# Autodesk Inventor assembly: Glue Stamp Staging Plate Assembly
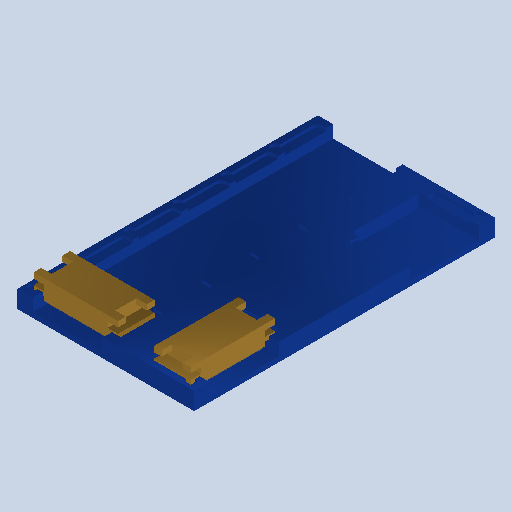
[picture p0: Inventor's stored thumbnail of the model, 512x512]
Saved by Autodesk Inventor 2022 (Build 260153000, 153)
## iProperties
Created: 2021-01-11
Part Number: Glue Stamp Staging Plate Assembly
Document SubType Name: Assembly
Designer: caleb
Author: caleb
## Documents named in this file (3)
- C:\Users\Caleb\Desktop\nebraska-silicon-lab\Hardware\ETL\Module Assembly\Glue Stamp Staging Plate\Glue Stamp Staging Plate Assembly.iam
- C:\Users\Caleb\Desktop\nebraska-silicon-lab\Hardware\ETL\Module Assembly\Glue Stamp Staging Plate\Glue Stamp Staging Plate.ipt
- C:\Users\Caleb\Desktop\nebraska-silicon-lab\Hardware\ETL\Module Assembly\Glue Stamp\Stamp Assembly.iam
## Components (3 placed, 2 different names)
1. Glue Stamp Staging Plate:1 — Mate:1, Mate:2, Mate:3, Mate:4, Mate:5, Mate:6
2. Stamp Assembly:1 [sub-assembly] — Mate:1, Mate:2, Mate:3
3. Stamp Assembly:2 [sub-assembly] — Mate:4, Mate:5, Mate:6
## Relationships (6: Mate 6)
- Mate:1: Glue Stamp Staging Plate:1 ↔ Stamp Assembly:1
- Mate:2: Glue Stamp Staging Plate:1 ↔ Stamp Assembly:1
- Mate:3: Glue Stamp Staging Plate:1 ↔ Stamp Assembly:1
- Mate:4: Glue Stamp Staging Plate:1 ↔ Stamp Assembly:2
- Mate:5: Glue Stamp Staging Plate:1 ↔ Stamp Assembly:2
- Mate:6: Glue Stamp Staging Plate:1 ↔ Stamp Assembly:2
